# Autodesk Inventor assembly: balloon_origin
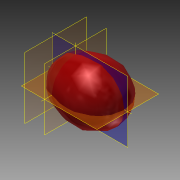
[picture p0: Inventor's stored thumbnail of the model, 180x180]
Saved by Autodesk Inventor 2015 (Build 190159000, 159)
## iProperties
Created: 2015-12-24
Part Number: balloon_origin
Document SubType Name: Assembly
Designer: Ryo
Author: Ryo
## Documents named in this file (2)
- D:\Users\Ryo\Documents\Inventor\motoman_cad\SIA5_TOOL\INVENTOR2015\balloon_origin.iam
- D:\Users\Ryo\Documents\Inventor\motoman_cad\SIA5_TOOL\INVENTOR2015\tool_3.ipt
## Components (1 placed, 1 different names)
1. tool_3:1 — フラッシュ:1, フラッシュ:2, 正接:1
## Relationships (3: Flush 2, Tangent 1)
- フラッシュ:1 [Flush]: tool_3:1
- フラッシュ:2 [Flush]: tool_3:1
- 正接:1 [Tangent]: tool_3:1
